# Autodesk Inventor assembly: DTraining2_001_E1Assembly
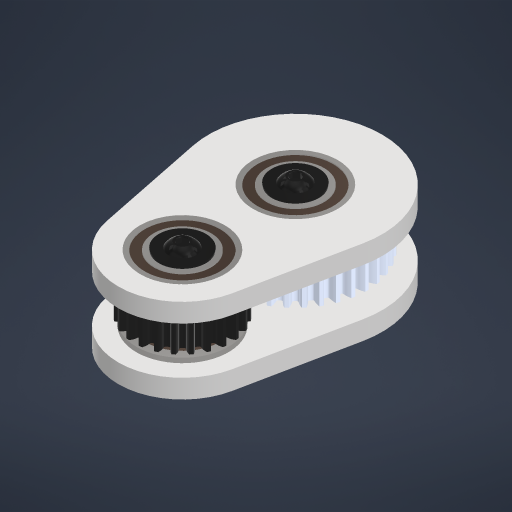
[picture p0: Inventor's stored thumbnail of the model, 512x512]
Saved by Autodesk Inventor 2024.4 (Build 284460000, 460)
## iProperties
Created: 2026-06-14
Part Number: DTraining2_001_E1Assembly
Document SubType Name: Assembly
Designer: hs4ho
Author: hs4ho
## Documents named in this file (7)
- C:\Users\hs4ho\OneDrive\Documents\GitHub\2026-2027-DesignTraining\DeanS\Design Training\DTraining2_001_E1Assembly.iam
- C:\Users\hs4ho\OneDrive\Documents\GitHub\2026-2027-DesignTraining\DeanS\Design Training\DTraining2_001_E1Base.ipt
- C:\Users\hs4ho\OneDrive\Documents\GitHub\2026-2027-DesignTraining\COTS Library\Motion\Bearings\COTS_WCP-0783_1.125ODHexBearing.ipt
- C:\Users\hs4ho\OneDrive\Documents\GitHub\2026-2027-DesignTraining\COTS Library\Motion\Gears\20DP gears\Aluminum\COTS_WCP-0703_24T_0.5inHex.ipt
- C:\Users\hs4ho\Downloads\WCP-0709\WCP-0709\WCP-0709.ipt
- C:\Users\hs4ho\OneDrive\Documents\GitHub\2026-2027-DesignTraining\DeanS\Design Training\DTraining2_001_E1Shaft.ipt
- C:\Users\hs4ho\OneDrive\Documents\GitHub\2026-2027-DesignTraining\COTS Library\Fasteners\Bolts\COTS_REV-21-2056_ShaftEndScrew_.5in.ipt
## Components (14 placed, 6 different names)
1. DTraining2_001_E1Base:1 — Mate:1, Mate:2, Mate:5, Mate:6, Mate:9, Mate:10
2. DTraining2_001_E1Base:2 — Mate:1, Mate:2, Mate:3, Mate:4, Mate:7, Mate:8
3. COTS_WCP-0783_1.125ODHexBearing:1 — Mate:3, Mate:4, Mate:13, Mate:16, Angle:3, Flush:1
4. COTS_WCP-0783_1.125ODHexBearing:2 — Mate:5, Mate:6, Mate:11, Angle:1, Mate:12
5. COTS_WCP-0783_1.125ODHexBearing:3 — Mate:7, Mate:8, Angle:2, Mate:15, Mate:17, Angle:4, Flush:2
6. COTS_WCP-0783_1.125ODHexBearing:4 — Mate:9, Mate:10, Mate:14, Angle:5
7. COTS_WCP-0703_24T_0.5inHex:1 — Mate:11, Angle:1, Mate:12, Mate:13, Angle:7
8. WCP-0709:1 — Mate:14, Angle:2, Mate:15
9. DTraining2_001_E1Shaft:1 — Mate:16, Angle:3, Flush:1, Mate:18, Mate:19, Angle:6, Angle:7, Mate:20, Mate:21, Angle:8
10. DTraining2_001_E1Shaft:2 — Mate:17, Angle:4, Flush:2, Angle:5, Mate:22, Mate:23, Angle:9, Mate:24, Mate:25, Angle:10
11. COTS_REV-21-2056_ShaftEndScrew_.5in:1 — Mate:18, Mate:19, Angle:6
12. COTS_REV-21-2056_ShaftEndScrew_.5in:2 — Mate:24, Mate:25, Angle:10
13. COTS_REV-21-2056_ShaftEndScrew_.5in:3 — Mate:22, Mate:23, Angle:9
14. COTS_REV-21-2056_ShaftEndScrew_.5in:4 — Mate:20, Mate:21, Angle:8
## Relationships (37: Mate 25, Angle 10, Flush 2)
- Mate:1: DTraining2_001_E1Base:1 ↔ DTraining2_001_E1Base:2
- Mate:2: DTraining2_001_E1Base:1 ↔ DTraining2_001_E1Base:2
- Mate:3: DTraining2_001_E1Base:2 ↔ COTS_WCP-0783_1.125ODHexBearing:1
- Mate:4: DTraining2_001_E1Base:2 ↔ COTS_WCP-0783_1.125ODHexBearing:1
- Mate:5: DTraining2_001_E1Base:1 ↔ COTS_WCP-0783_1.125ODHexBearing:2
- Mate:6: DTraining2_001_E1Base:1 ↔ COTS_WCP-0783_1.125ODHexBearing:2
- Mate:7: DTraining2_001_E1Base:2 ↔ COTS_WCP-0783_1.125ODHexBearing:3
- Mate:8: DTraining2_001_E1Base:2 ↔ COTS_WCP-0783_1.125ODHexBearing:3
- Mate:9: DTraining2_001_E1Base:1 ↔ COTS_WCP-0783_1.125ODHexBearing:4
- Mate:10: DTraining2_001_E1Base:1 ↔ COTS_WCP-0783_1.125ODHexBearing:4
- Mate:11: COTS_WCP-0783_1.125ODHexBearing:2 ↔ COTS_WCP-0703_24T_0.5inHex:1
- Angle:1 (0 deg): COTS_WCP-0783_1.125ODHexBearing:2 ↔ COTS_WCP-0703_24T_0.5inHex:1
- Mate:12: COTS_WCP-0783_1.125ODHexBearing:2 ↔ COTS_WCP-0703_24T_0.5inHex:1
- Mate:13: COTS_WCP-0783_1.125ODHexBearing:1 ↔ COTS_WCP-0703_24T_0.5inHex:1
- Mate:14: COTS_WCP-0783_1.125ODHexBearing:4 ↔ WCP-0709:1
- Angle:2 (0 deg): COTS_WCP-0783_1.125ODHexBearing:3 ↔ WCP-0709:1
- Mate:15: COTS_WCP-0783_1.125ODHexBearing:3 ↔ WCP-0709:1
- Mate:16: COTS_WCP-0783_1.125ODHexBearing:1 ↔ DTraining2_001_E1Shaft:1
- Angle:3 (0 deg): COTS_WCP-0783_1.125ODHexBearing:1 ↔ DTraining2_001_E1Shaft:1
- Flush:1: COTS_WCP-0783_1.125ODHexBearing:1 ↔ DTraining2_001_E1Shaft:1
- Mate:17: COTS_WCP-0783_1.125ODHexBearing:3 ↔ DTraining2_001_E1Shaft:2
- Angle:4 (0 deg): COTS_WCP-0783_1.125ODHexBearing:3 ↔ DTraining2_001_E1Shaft:2
- Flush:2: COTS_WCP-0783_1.125ODHexBearing:3 ↔ DTraining2_001_E1Shaft:2
- Angle:5 (0 deg): COTS_WCP-0783_1.125ODHexBearing:4 ↔ DTraining2_001_E1Shaft:2
- Mate:18: DTraining2_001_E1Shaft:1 ↔ COTS_REV-21-2056_ShaftEndScrew_.5in:1
- Mate:19: DTraining2_001_E1Shaft:1 ↔ COTS_REV-21-2056_ShaftEndScrew_.5in:1
- Angle:6 (0 deg): DTraining2_001_E1Shaft:1 ↔ COTS_REV-21-2056_ShaftEndScrew_.5in:1
- Angle:7 (0 deg): COTS_WCP-0703_24T_0.5inHex:1 ↔ DTraining2_001_E1Shaft:1
- Mate:20: DTraining2_001_E1Shaft:1 ↔ COTS_REV-21-2056_ShaftEndScrew_.5in:4
- Mate:21: DTraining2_001_E1Shaft:1 ↔ COTS_REV-21-2056_ShaftEndScrew_.5in:4
- Angle:8 (0 deg): DTraining2_001_E1Shaft:1 ↔ COTS_REV-21-2056_ShaftEndScrew_.5in:4
- Mate:22: DTraining2_001_E1Shaft:2 ↔ COTS_REV-21-2056_ShaftEndScrew_.5in:3
- Mate:23: DTraining2_001_E1Shaft:2 ↔ COTS_REV-21-2056_ShaftEndScrew_.5in:3
- Angle:9 (0 deg): DTraining2_001_E1Shaft:2 ↔ COTS_REV-21-2056_ShaftEndScrew_.5in:3
- Mate:24: DTraining2_001_E1Shaft:2 ↔ COTS_REV-21-2056_ShaftEndScrew_.5in:2
- Mate:25: DTraining2_001_E1Shaft:2 ↔ COTS_REV-21-2056_ShaftEndScrew_.5in:2
- Angle:10 (0 deg): DTraining2_001_E1Shaft:2 ↔ COTS_REV-21-2056_ShaftEndScrew_.5in:2
